# Autodesk Inventor assembly: Leg
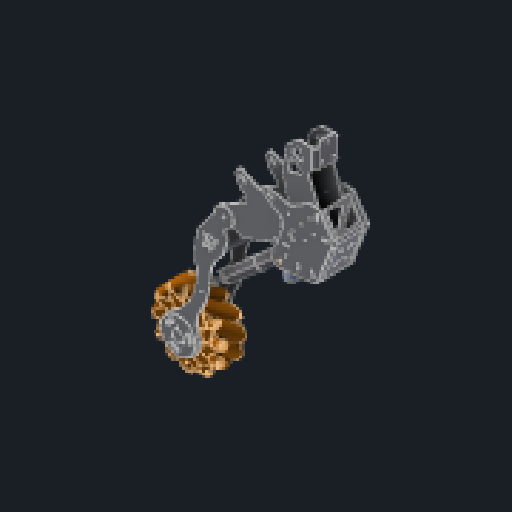
[picture p0: Inventor's stored thumbnail of the model, 512x512]
Saved by Autodesk Inventor 2025.2 (Build 292293000, 293)
## iProperties
_SolveAssemblyDoc: Frame Generator Solve Assembly
_Version: 15.0.0
Created: 2020-05-17
Part Number: Leg
Document SubType Name: Assembly
Designer: valer
Author: valer
## Documents named in this file (17)
- C:\Users\valer\Desktop\str1ker\cad\Leg.iam
- C:\Users\valer\Desktop\str1ker\cad\LegThigh.ipt
- C:\Users\valer\Desktop\str1ker\cad\LegShin.ipt
- C:\Users\valer\Desktop\str1ker\cad\LegHipSide.ipt
- C:\Users\valer\Desktop\str1ker\cad\LegHip.ipt
- C:\Users\valer\Desktop\str1ker\cad\LegHipFront.ipt
- C:\Users\valer\Desktop\str1ker\cad\external\2796N15_Omni-Directional Wheel.ipt
- C:\Users\valer\Desktop\str1ker\cad\external\MY6812-12VDC-120W-Motor.ipt
- C:\Users\valer\Desktop\str1ker\cad\external\SprocketMDEOOSKY-25H-47T.ipt
- C:\Users\valer\Desktop\str1ker\cad\LegHub.ipt
- C:\Users\valer\Desktop\str1ker\cad\external\6656K234_Ultra-Thin Ball Bearing.ipt
- C:\Users\valer\Desktop\str1ker\cad\LegInsideConnector.ipt
- C:\Users\valer\Desktop\str1ker\cad\external\FA-RMS-15-12-4.ipt
- C:\Users\valer\Desktop\str1ker\cad\external\FA-RMS-15-12-4-Piston.ipt
- C:\Users\valer\Desktop\str1ker\cad\external\np32hs.iam
- C:\Users\valer\Desktop\str1ker\cad\LegHandleDesign.ipt
- C:\Users\valer\Desktop\str1ker\cad\LegHandle.iam
## Components (22 placed, 16 different names)
1. LegThigh:1 — Flush:1, Mate:1, Mate:4, Mate:112
2. LegHipSide:1 — Flush:1, Mate:1, Mate:4, Mate:6, Mate:7, Symmetry:1, Mate:137, Mate:140
3. LegHip:1 — Mate:6, Mate:7, Flush:6, Mate:134, Mate:135, Mate:141
4. LegThigh:2 — Mate:115, Mate:130, Mate:131, Mate:133, Flush:137, Mate:136, Mate:139
5. LegHipSide:2 — Symmetry:1, Mate:124
6. LegHipFront:1 — Angle:2, Mate:140
7. MY6812-12VDC-120W-Motor:1 — Mate:77, Mate:80, Mate:89, Mate:93, Flush:4, Flush:5, Mate:132
8. LegShin:3 — Mate:77, Mate:80, Mate:94
9. LegShin:4 — Mate:89, Mate:98, Mate:111, Mate:127, Mate:132, Mate:133, Angle:1, Mate:139
10. SprocketMDEOOSKY-25H-47T:1 — Flush:4, Mate:96, Mate:110, Flush:5
11. LegHub:1 — Mate:94, Mate:97, Mate:108, Mate:109, Mate:110
12. 2796N15_Omni-Directional Wheel:1 — Mate:96, Mate:97, Mate:98, Mate:102, Mate:103, Mate:104, Mate:105, Mate:106, Mate:107, Mate:108, Mate:109
13. 6656K234_Ultra-Thin Ball Bearing:1 — Mate:102, Mate:111
14. 6656K234_Ultra-Thin Ball Bearing:2 — Mate:103, Mate:104
15. LegHub:3 — Mate:105, Mate:106, Mate:107
16. LegInsideConnector:1 — Mate:112
17. LegInsideConnector:2 — Mate:115, Mate:130, Mate:131, Mate:141
18. FA-RMS-15-12-4:1 — Mate:124, Mate:125, Mate:126
19. FA-RMS-15-12-4-Piston:1 — Mate:126, Mate:127
20. np32hs:1 [sub-assembly] — Flush:137, Mate:136, Angle:1
21. LegHandleDesign:1 — Flush:138, Mate:138
22. LegHandle:1 [sub-assembly]
## Relationships (50: Mate 40, Flush 7, Angle 2, Symmetry 1)
- Flush:1 (-5.08 mm): LegThigh:1 ↔ LegHipSide:1
- Mate:1: LegThigh:1 ↔ LegHipSide:1
- Mate:4: LegThigh:1 ↔ LegHipSide:1
- Mate:6: LegHipSide:1 ↔ LegHip:1
- Mate:7: LegHipSide:1 ↔ LegHip:1
- [Flush] (5.08 mm): LegThigh:2 ↔ LegHipSide:2
- Symmetry:1: LegHipSide:1 ↔ LegHipSide:2
- Mate:77: MY6812-12VDC-120W-Motor:1 ↔ LegShin:3
- Mate:80: MY6812-12VDC-120W-Motor:1 ↔ LegShin:3
- Mate:89: MY6812-12VDC-120W-Motor:1 ↔ LegShin:4
- Mate:93: MY6812-12VDC-120W-Motor:1
- Mate:94: LegShin:3 ↔ LegHub:1
- Flush:4: MY6812-12VDC-120W-Motor:1 ↔ SprocketMDEOOSKY-25H-47T:1
- Mate:96: SprocketMDEOOSKY-25H-47T:1 ↔ 2796N15_Omni-Directional Wheel:1
- Mate:97: LegHub:1 ↔ 2796N15_Omni-Directional Wheel:1
- Mate:98: LegShin:4 ↔ 2796N15_Omni-Directional Wheel:1
- Mate:102: 2796N15_Omni-Directional Wheel:1 ↔ 6656K234_Ultra-Thin Ball Bearing:1
- Mate:103: 2796N15_Omni-Directional Wheel:1 ↔ 6656K234_Ultra-Thin Ball Bearing:2
- Mate:104: 2796N15_Omni-Directional Wheel:1 ↔ 6656K234_Ultra-Thin Ball Bearing:2
- Mate:105: 2796N15_Omni-Directional Wheel:1 ↔ LegHub:3
- Mate:106: 2796N15_Omni-Directional Wheel:1 ↔ LegHub:3
- Mate:107: 2796N15_Omni-Directional Wheel:1 ↔ LegHub:3
- Mate:108: LegHub:1 ↔ 2796N15_Omni-Directional Wheel:1
- Mate:109: LegHub:1 ↔ 2796N15_Omni-Directional Wheel:1
- Mate:110: SprocketMDEOOSKY-25H-47T:1 ↔ LegHub:1
- Flush:5: MY6812-12VDC-120W-Motor:1 ↔ SprocketMDEOOSKY-25H-47T:1
- Mate:111: LegShin:4 ↔ 6656K234_Ultra-Thin Ball Bearing:1
- Mate:112: LegThigh:1 ↔ LegInsideConnector:1
- Mate:115: LegThigh:2 ↔ LegInsideConnector:2
- Mate:124: LegHipSide:2 ↔ FA-RMS-15-12-4:1
- Mate:125: FA-RMS-15-12-4:1
- Mate:126: FA-RMS-15-12-4:1 ↔ FA-RMS-15-12-4-Piston:1
- Mate:127: LegShin:4 ↔ FA-RMS-15-12-4-Piston:1
- Flush:6: LegHip:1
- Mate:130: LegThigh:2 ↔ LegInsideConnector:2
- Mate:131: LegThigh:2 ↔ LegInsideConnector:2
- Mate:132: MY6812-12VDC-120W-Motor:1 ↔ LegShin:4
- Mate:133: LegThigh:2 ↔ LegShin:4
- Mate:134: LegHip:1
- Mate:135: LegHip:1
- Flush:137: LegThigh:2 ↔ np32hs:1
- Mate:136: LegThigh:2 ↔ np32hs:1
- Angle:1 (0 deg): LegShin:4 ↔ np32hs:1
- Mate:137: LegHipSide:1
- Angle:2 (0 deg): LegHipFront:1
- Flush:138: LegHandleDesign:1
- Mate:138: LegHandleDesign:1
- Mate:139: LegThigh:2 ↔ LegShin:4
- Mate:140: LegHipSide:1 ↔ LegHipFront:1
- Mate:141: LegHip:1 ↔ LegInsideConnector:2
## Named parameters: d11_d0 = 5.08 mm
